# Autodesk Inventor assembly: NEO Turn Gear
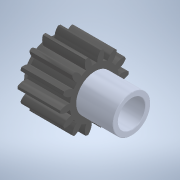
[picture p0: Inventor's stored thumbnail of the model, 180x180]
Saved by Autodesk Inventor 2023 (Build 270158000, 158)
## iProperties
Created: 2023-03-28
Part Number: NEO Turn Gear
Document SubType Name: Assembly
Designer: jackc
Author: jackc
## Documents named in this file (5)
- G:\.shortcut-targets-by-id\1MkDWIt6nIPqRnJSGLfoCUaNz0aFopGUn\1939_Arnold\2_Design\2023-2024\Parts\Swerve\NEO Drive Gear.iam
- G:\.shortcut-targets-by-id\1MkDWIt6nIPqRnJSGLfoCUaNz0aFopGUn\1939_Arnold\2_Design\2023-2024\Parts\Swerve\Gear, 20DP, 14T, 8mm REV1.ipt
- G:\.shortcut-targets-by-id\1MkDWIt6nIPqRnJSGLfoCUaNz0aFopGUn\1939_Arnold\2_Design\2023-2024\Parts\Swerve\Retaining Ring, 8mm, 98430A132.ipt
- G:\.shortcut-targets-by-id\1MkDWIt6nIPqRnJSGLfoCUaNz0aFopGUn\1939_Arnold\2_Design\2023-2024\Parts\Swerve\Machine Key, 2 X 2 X 12mm.ipt
- G:\.shortcut-targets-by-id\1MkDWIt6nIPqRnJSGLfoCUaNz0aFopGUn\1939_Arnold\2_Design\2023-2024\Parts\Swerve\Spacer, 8mmID X .437 OD X 0.437 L.ipt
## Components (4 placed, 4 different names)
1. Gear, 20DP, 14T, 8mm REV1:1 — Insert:1, Mate:1, Mate:2, Insert:2, Tangent:1
2. Retaining Ring, 8mm, 98430A132:1 — Insert:1
3. Machine Key, 2 X 2 X 12mm:1 — Mate:1, Mate:2, Tangent:1
4. Spacer, 8mmID X .437 OD X 0.437 L:1 — Insert:2
## Relationships (5: Insert 2, Mate 2, Tangent 1)
- Insert:1: Gear, 20DP, 14T, 8mm REV1:1 ↔ Retaining Ring, 8mm, 98430A132:1
- Mate:1: Gear, 20DP, 14T, 8mm REV1:1 ↔ Machine Key, 2 X 2 X 12mm:1
- Mate:2: Gear, 20DP, 14T, 8mm REV1:1 ↔ Machine Key, 2 X 2 X 12mm:1
- Insert:2: Gear, 20DP, 14T, 8mm REV1:1 ↔ Spacer, 8mmID X .437 OD X 0.437 L:1
- Tangent:1: Gear, 20DP, 14T, 8mm REV1:1 ↔ Machine Key, 2 X 2 X 12mm:1
